# Autodesk Inventor assembly: 200-40-BOGIE-CONNECTOR-ASM-01
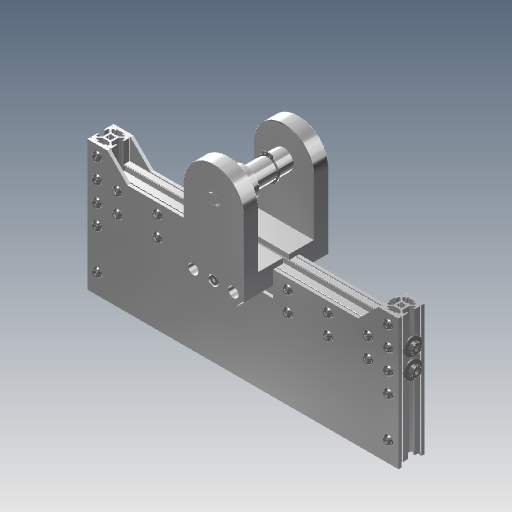
[picture p0: Inventor's stored thumbnail of the model, 512x512]
Saved by Autodesk Inventor 2018.2 (Build 222227000, 227)
## iProperties
Manager: feesmrt
Company: FRANC0R
Created: 2017-12-10
Part Number: 200-40-BOGIE-CONNECTOR-ASM-01
Material: Generisch
Document SubType Name: Assembly
Designer: feesmrt
Project: Rescue Robot
Cost Center: -
Description: Bogie Connector Assembly
Engineer: feesmrt
Authority: feesmrt
Stock Number: 200-40-BOGIE-CONNECTOR-ASM-01
Mass: 975.454 g
Surface Area: 1626.6 cm^2
Volume: 351.256 cm^3
Density: 2.77705 g/cm^3
Author: feesmrt
Title: Bogie Connector Assembly
Subject: Rescue Robot
Revision Number: 1
## Documents named in this file (13)
- D:\Programmierung\FRANC0R\CAD\02-Rocker-Bogie-Robot\200-ROCKER-BOGIE\200-40-BOGIE-CONNECTOR\200-40-BOGIE-CONNECTOR-ASM-01.iam
- D:\Programmierung\FRANC0R\CAD\02-Rocker-Bogie-Robot\200-ROCKER-BOGIE\200-40-BOGIE-CONNECTOR\200-40-BOGIE-CONNECTOR-05.ipt
- D:\Programmierung\FRANC0R\CAD\02-Rocker-Bogie-Robot\200-ROCKER-BOGIE\200-40-BOGIE-CONNECTOR\200-40-BOGIE-CONNECTOR-03.ipt
- D:\Programmierung\FRANC0R\CAD\02-Rocker-Bogie-Robot\200-ROCKER-BOGIE\200-40-BOGIE-CONNECTOR\200-40-BOGIE-CONNECTOR-04.ipt
- D:\Programmierung\FRANC0R\CAD\02-Rocker-Bogie-Robot\900-COMPONENTS\900-40-SCREWS\900-40-SCREWS-DIN7984_M5x25.ipt
- D:\Programmierung\FRANC0R\CAD\02-Rocker-Bogie-Robot\900-COMPONENTS\900-40-SCREWS\900-40-SCREWS-DIN7984_M5x12.ipt
- D:\Programmierung\FRANC0R\CAD\02-Rocker-Bogie-Robot\900-COMPONENTS\900-50-PROFILES\900-50-PROFILES-CONN-N6xM5.ipt
- D:\Programmierung\FRANC0R\CAD\02-Rocker-Bogie-Robot\900-COMPONENTS\900-60-CIRCLIPS\900-60-CIRCLIPS-DIN471-20x1,2.ipt
- D:\Programmierung\FRANC0R\CAD\02-Rocker-Bogie-Robot\200-ROCKER-BOGIE\200-40-BOGIE-CONNECTOR\200-40-BOGIE-CONNECTOR-P-01.ipt
- D:\Programmierung\FRANC0R\CAD\02-Rocker-Bogie-Robot\200-ROCKER-BOGIE\200-40-BOGIE-CONNECTOR\200-40-BOGIE-CONNECTOR-P-02.ipt
- D:\Programmierung\FRANC0R\CAD\02-Rocker-Bogie-Robot\200-ROCKER-BOGIE\200-40-BOGIE-CONNECTOR\200-40-BOGIE-CONNECTOR-REINFORCEMENT-01.iam
- D:\Programmierung\FRANC0R\CAD\02-Rocker-Bogie-Robot\900-COMPONENTS\900-80-WASHERS\900-80-WASHERS-DIN9021-M6.ipt
- D:\Programmierung\FRANC0R\CAD\02-Rocker-Bogie-Robot\900-COMPONENTS\900-40-SCREWS\900-40-SCREWS-DIN7984_M6x30.ipt
## Components (29 placed, 12 different names)
1. 200-40-BOGIE-CONNECTOR-05:1 — Passend:6, Passend:7, Fluchtend:7, Passend:8, Passend:9, Passend:10, Passend:45, Passend:46
2. 200-40-BOGIE-CONNECTOR-03:2 — Passend:8, Passend:9, Passend:10, Passend:16, Fluchtend:10, Passend:23, Passend:25, Passend:34, Passend:35
3. 200-40-BOGIE-CONNECTOR-03:1 — Passend:6, Passend:7, Fluchtend:7, Passend:17, Passend:24, Fluchtend:11, Passend:33, Passend:36
4. 200-40-BOGIE-CONNECTOR-04:1 — Passend:17, Passend:24, Fluchtend:11, Passend:29, Passend:30, Passend:31, Passend:32, Passend:39, Passend:40, Winkel:1, Winkel:2, Passend:49
5. 200-40-BOGIE-CONNECTOR-04:2 — Passend:16, Fluchtend:10, Passend:23, Passend:26, Passend:27, Passend:28, Passend:37, Passend:38, Winkel:3, Winkel:4
6. 900-40-SCREWS-DIN7984_M5x25:1 — Passend:25, Passend:26, Passend:41
7. 900-40-SCREWS-DIN7984_M5x25:2 — Passend:27, Passend:28, Passend:42
8. 900-40-SCREWS-DIN7984_M5x25:3 — Passend:30, Passend:32, Passend:44
9. 900-40-SCREWS-DIN7984_M5x25:4 — Passend:29, Passend:31, Passend:43
10. 900-40-SCREWS-DIN7984_M5x12:1 — Passend:33, Passend:36
11. 900-40-SCREWS-DIN7984_M5x12:2 — Passend:34, Passend:35
12. 900-50-PROFILES-CONN-N6xM5:1 — Passend:37, Passend:42, Winkel:4
13. 900-50-PROFILES-CONN-N6xM5:2 — Passend:38, Passend:41, Winkel:3
14. 900-50-PROFILES-CONN-N6xM5:3 — Passend:40, Passend:44, Winkel:2
15. 900-50-PROFILES-CONN-N6xM5:4 — Passend:39, Passend:43, Winkel:1
16. 900-60-CIRCLIPS-DIN471-20x1,2:1 — Passend:45, Passend:46, Fluchtend:12
17. 200-40-BOGIE-CONNECTOR-P-01:1 — Passend:47, Passend:48, Passend:49, Fluchtend:13, Fluchtend:14, Fluchtend:15, Fluchtend:16, Passend:50, Passend:51, Passend:53, Passend:55, Passend:57
18. 200-40-BOGIE-CONNECTOR-P-02:1 — Fluchtend:13, Fluchtend:15, Passend:50, Passend:58, Passend:59, Passend:60, Passend:61
19. 200-40-BOGIE-CONNECTOR-P-02:2 — Fluchtend:14, Fluchtend:16, Passend:51, Passend:52, Passend:54, Passend:56, Passend:62, Passend:63, Passend:64, Passend:65
20. 200-40-BOGIE-CONNECTOR-REINFORCEMENT-01:1 [sub-assembly] — Passend:52, Passend:53, Passend:54
21. 200-40-BOGIE-CONNECTOR-REINFORCEMENT-01:2 [sub-assembly] — Passend:55, Passend:56, Passend:57
22. 900-80-WASHERS-DIN9021-M6:1 — Passend:58, Passend:60, Passend:66, Passend:72
23. 900-80-WASHERS-DIN9021-M6:2 — Passend:59, Passend:61, Passend:67, Passend:73
24. 900-80-WASHERS-DIN9021-M6:3 — Passend:62, Passend:65, Passend:69, Passend:70
25. 900-80-WASHERS-DIN9021-M6:4 — Passend:63, Passend:64, Passend:68, Passend:71
26. 900-40-SCREWS-DIN7984_M6x30:1 — Passend:66, Passend:72
27. 900-40-SCREWS-DIN7984_M6x30:2 — Passend:67, Passend:73
28. 900-40-SCREWS-DIN7984_M6x30:3 — Passend:69, Passend:70
29. 900-40-SCREWS-DIN7984_M6x30:4 — Passend:68, Passend:71
## Relationships (70: Mate 58, Flush 8, Angle 4)
- Passend:6 [Mate]: 200-40-BOGIE-CONNECTOR-05:1 ↔ 200-40-BOGIE-CONNECTOR-03:1
- Passend:7 [Mate]: 200-40-BOGIE-CONNECTOR-05:1 ↔ 200-40-BOGIE-CONNECTOR-03:1
- Fluchtend:7 [Flush]: 200-40-BOGIE-CONNECTOR-05:1 ↔ 200-40-BOGIE-CONNECTOR-03:1
- Passend:8 [Mate]: 200-40-BOGIE-CONNECTOR-05:1 ↔ 200-40-BOGIE-CONNECTOR-03:2
- Passend:9 [Mate]: 200-40-BOGIE-CONNECTOR-05:1 ↔ 200-40-BOGIE-CONNECTOR-03:2
- Passend:10 [Mate]: 200-40-BOGIE-CONNECTOR-05:1 ↔ 200-40-BOGIE-CONNECTOR-03:2
- Passend:16 [Mate]: 200-40-BOGIE-CONNECTOR-03:2 ↔ 200-40-BOGIE-CONNECTOR-04:2
- Passend:17 [Mate]: 200-40-BOGIE-CONNECTOR-03:1 ↔ 200-40-BOGIE-CONNECTOR-04:1
- Fluchtend:10 [Flush]: 200-40-BOGIE-CONNECTOR-03:2 ↔ 200-40-BOGIE-CONNECTOR-04:2
- Passend:23 [Mate]: 200-40-BOGIE-CONNECTOR-03:2 ↔ 200-40-BOGIE-CONNECTOR-04:2
- Passend:24 [Mate]: 200-40-BOGIE-CONNECTOR-03:1 ↔ 200-40-BOGIE-CONNECTOR-04:1
- Fluchtend:11 [Flush]: 200-40-BOGIE-CONNECTOR-03:1 ↔ 200-40-BOGIE-CONNECTOR-04:1
- Passend:25 [Mate]: 200-40-BOGIE-CONNECTOR-03:2 ↔ 900-40-SCREWS-DIN7984_M5x25:1
- Passend:26 [Mate]: 200-40-BOGIE-CONNECTOR-04:2 ↔ 900-40-SCREWS-DIN7984_M5x25:1
- Passend:27 [Mate]: 200-40-BOGIE-CONNECTOR-04:2 ↔ 900-40-SCREWS-DIN7984_M5x25:2
- Passend:28 [Mate]: 200-40-BOGIE-CONNECTOR-04:2 ↔ 900-40-SCREWS-DIN7984_M5x25:2
- Passend:29 [Mate]: 200-40-BOGIE-CONNECTOR-04:1 ↔ 900-40-SCREWS-DIN7984_M5x25:4
- Passend:30 [Mate]: 200-40-BOGIE-CONNECTOR-04:1 ↔ 900-40-SCREWS-DIN7984_M5x25:3
- Passend:31 [Mate]: 200-40-BOGIE-CONNECTOR-04:1 ↔ 900-40-SCREWS-DIN7984_M5x25:4
- Passend:32 [Mate]: 200-40-BOGIE-CONNECTOR-04:1 ↔ 900-40-SCREWS-DIN7984_M5x25:3
- Passend:33 [Mate]: 200-40-BOGIE-CONNECTOR-03:1 ↔ 900-40-SCREWS-DIN7984_M5x12:1
- Passend:34 [Mate]: 200-40-BOGIE-CONNECTOR-03:2 ↔ 900-40-SCREWS-DIN7984_M5x12:2
- Passend:35 [Mate]: 200-40-BOGIE-CONNECTOR-03:2 ↔ 900-40-SCREWS-DIN7984_M5x12:2
- Passend:36 [Mate]: 200-40-BOGIE-CONNECTOR-03:1 ↔ 900-40-SCREWS-DIN7984_M5x12:1
- Passend:37 [Mate] (1.5 mm): 200-40-BOGIE-CONNECTOR-04:2 ↔ 900-50-PROFILES-CONN-N6xM5:1
- Passend:38 [Mate] (1.5 mm): 200-40-BOGIE-CONNECTOR-04:2 ↔ 900-50-PROFILES-CONN-N6xM5:2
- Passend:39 [Mate] (1.5 mm): 200-40-BOGIE-CONNECTOR-04:1 ↔ 900-50-PROFILES-CONN-N6xM5:4
- Passend:40 [Mate] (1.5 mm): 200-40-BOGIE-CONNECTOR-04:1 ↔ 900-50-PROFILES-CONN-N6xM5:3
- Passend:41 [Mate]: 900-40-SCREWS-DIN7984_M5x25:1 ↔ 900-50-PROFILES-CONN-N6xM5:2
- Passend:42 [Mate]: 900-40-SCREWS-DIN7984_M5x25:2 ↔ 900-50-PROFILES-CONN-N6xM5:1
- Passend:43 [Mate]: 900-40-SCREWS-DIN7984_M5x25:4 ↔ 900-50-PROFILES-CONN-N6xM5:4
- Passend:44 [Mate]: 900-40-SCREWS-DIN7984_M5x25:3 ↔ 900-50-PROFILES-CONN-N6xM5:3
- Winkel:1 [Angle] (0 deg): 200-40-BOGIE-CONNECTOR-04:1 ↔ 900-50-PROFILES-CONN-N6xM5:4
- Winkel:2 [Angle] (0 deg): 200-40-BOGIE-CONNECTOR-04:1 ↔ 900-50-PROFILES-CONN-N6xM5:3
- Winkel:3 [Angle] (0 deg): 200-40-BOGIE-CONNECTOR-04:2 ↔ 900-50-PROFILES-CONN-N6xM5:2
- Winkel:4 [Angle] (0 deg): 200-40-BOGIE-CONNECTOR-04:2 ↔ 900-50-PROFILES-CONN-N6xM5:1
- Passend:45 [Mate]: 200-40-BOGIE-CONNECTOR-05:1 ↔ 900-60-CIRCLIPS-DIN471-20x1,2:1
- Passend:46 [Mate]: 200-40-BOGIE-CONNECTOR-05:1 ↔ 900-60-CIRCLIPS-DIN471-20x1,2:1
- Fluchtend:12 [Flush]: 900-60-CIRCLIPS-DIN471-20x1,2:1
- Passend:47 [Mate]: 200-40-BOGIE-CONNECTOR-P-01:1
- Passend:48 [Mate]: 200-40-BOGIE-CONNECTOR-P-01:1
- Passend:49 [Mate]: 200-40-BOGIE-CONNECTOR-04:1 ↔ 200-40-BOGIE-CONNECTOR-P-01:1
- Fluchtend:13 [Flush] (-20 mm): 200-40-BOGIE-CONNECTOR-P-01:1 ↔ 200-40-BOGIE-CONNECTOR-P-02:1
- Fluchtend:14 [Flush] (-20 mm): 200-40-BOGIE-CONNECTOR-P-01:1 ↔ 200-40-BOGIE-CONNECTOR-P-02:2
- Fluchtend:15 [Flush]: 200-40-BOGIE-CONNECTOR-P-01:1 ↔ 200-40-BOGIE-CONNECTOR-P-02:1
- Fluchtend:16 [Flush]: 200-40-BOGIE-CONNECTOR-P-01:1 ↔ 200-40-BOGIE-CONNECTOR-P-02:2
- Passend:50 [Mate]: 200-40-BOGIE-CONNECTOR-P-01:1 ↔ 200-40-BOGIE-CONNECTOR-P-02:1
- Passend:51 [Mate]: 200-40-BOGIE-CONNECTOR-P-01:1 ↔ 200-40-BOGIE-CONNECTOR-P-02:2
- Passend:52 [Mate]: 200-40-BOGIE-CONNECTOR-P-02:2 ↔ 200-40-BOGIE-CONNECTOR-REINFORCEMENT-01:1
- Passend:53 [Mate]: 200-40-BOGIE-CONNECTOR-P-01:1 ↔ 200-40-BOGIE-CONNECTOR-REINFORCEMENT-01:1
- Passend:54 [Mate]: 200-40-BOGIE-CONNECTOR-P-02:2 ↔ 200-40-BOGIE-CONNECTOR-REINFORCEMENT-01:1
- Passend:55 [Mate]: 200-40-BOGIE-CONNECTOR-P-01:1 ↔ 200-40-BOGIE-CONNECTOR-REINFORCEMENT-01:2
- Passend:56 [Mate]: 200-40-BOGIE-CONNECTOR-P-02:2 ↔ 200-40-BOGIE-CONNECTOR-REINFORCEMENT-01:2
- Passend:57 [Mate]: 200-40-BOGIE-CONNECTOR-P-01:1 ↔ 200-40-BOGIE-CONNECTOR-REINFORCEMENT-01:2
- Passend:58 [Mate]: 200-40-BOGIE-CONNECTOR-P-02:1 ↔ 900-80-WASHERS-DIN9021-M6:1
- Passend:59 [Mate]: 200-40-BOGIE-CONNECTOR-P-02:1 ↔ 900-80-WASHERS-DIN9021-M6:2
- Passend:60 [Mate]: 200-40-BOGIE-CONNECTOR-P-02:1 ↔ 900-80-WASHERS-DIN9021-M6:1
- Passend:61 [Mate]: 200-40-BOGIE-CONNECTOR-P-02:1 ↔ 900-80-WASHERS-DIN9021-M6:2
- Passend:62 [Mate]: 200-40-BOGIE-CONNECTOR-P-02:2 ↔ 900-80-WASHERS-DIN9021-M6:3
- Passend:63 [Mate]: 200-40-BOGIE-CONNECTOR-P-02:2 ↔ 900-80-WASHERS-DIN9021-M6:4
- Passend:64 [Mate]: 200-40-BOGIE-CONNECTOR-P-02:2 ↔ 900-80-WASHERS-DIN9021-M6:4
- Passend:65 [Mate]: 200-40-BOGIE-CONNECTOR-P-02:2 ↔ 900-80-WASHERS-DIN9021-M6:3
- Passend:66 [Mate]: 900-80-WASHERS-DIN9021-M6:1 ↔ 900-40-SCREWS-DIN7984_M6x30:1
- Passend:67 [Mate]: 900-80-WASHERS-DIN9021-M6:2 ↔ 900-40-SCREWS-DIN7984_M6x30:2
- Passend:68 [Mate]: 900-80-WASHERS-DIN9021-M6:4 ↔ 900-40-SCREWS-DIN7984_M6x30:4
- Passend:69 [Mate]: 900-80-WASHERS-DIN9021-M6:3 ↔ 900-40-SCREWS-DIN7984_M6x30:3
- Passend:70 [Mate]: 900-80-WASHERS-DIN9021-M6:3 ↔ 900-40-SCREWS-DIN7984_M6x30:3
- Passend:71 [Mate]: 900-80-WASHERS-DIN9021-M6:4 ↔ 900-40-SCREWS-DIN7984_M6x30:4
- Passend:72 [Mate]: 900-80-WASHERS-DIN9021-M6:1 ↔ 900-40-SCREWS-DIN7984_M6x30:1
- Passend:73 [Mate]: 900-80-WASHERS-DIN9021-M6:2 ↔ 900-40-SCREWS-DIN7984_M6x30:2
